# Autodesk Inventor assembly: DeviceForScheme
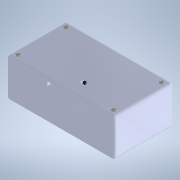
[picture p0: Inventor's stored thumbnail of the model, 180x180]
Saved by Autodesk Inventor 2022 (Build 260153000, 153)
## iProperties
Created: 2021-03-07
Part Number: DeviceForScheme
Description: STEP AP214
Document SubType Name: Assembly
Designer: user
Sending System: SolidWorks 2017
Preprocessor: SwSTEP 2.0
Title: Gainta G1098.STEP
Revision Number: ANY
## Documents named in this file (6)
- C:\Study\Diplom\case\DeviceForScheme.iam
- C:\Study\Diplom\case\Îñíîâàíèå.ipt
- C:\Study\Diplom\case\Êðûøêà.ipt
- C:\Study\Diplom\Altium\Diplom\Project Outputs for Diplom\InventorNew\PCBDiplomPCB.iam
- C:\Users\user\Documents\Inventor\Content Center Files\R2022\ru-RU\AS 1427(05)\AS 1427 - M2.5 x 16(5) II.ipt
- C:\Users\user\Documents\Inventor\Content Center Files\R2022\ru-RU\AS 1427(05)\AS 1427 - M3 x 5(5) II.ipt
## Components (11 placed, 5 different names)
1. Îñíîâàíèå_1 — Вставка:6
2. Êðûøêà_2 — Вставка:1, Вставка:4, Вставка:5, Вставка:6, Вставка:7, Вставка:8, Вставка:9, Вставка:10
3. PCBDiplomPCB:1 [sub-assembly] — Вставка:1, Вставка:2, Вставка:3
4. AS 1427 H - метрическая M2.5 x 16:1 — Вставка:8
5. AS 1427 H - метрическая M2.5 x 16:2 — Вставка:9
6. AS 1427 H - метрическая M2.5 x 16:3 — Вставка:7
7. AS 1427 H - метрическая M2.5 x 16:4 — Вставка:10
8. AS 1427 H - метрическая M3 x 5:1 — Вставка:3
9. AS 1427 H - метрическая M3 x 5:2 — Вставка:4
10. AS 1427 H - метрическая M3 x 5:3 — Вставка:5
11. AS 1427 H - метрическая M3 x 5:4 — Вставка:2
## Relationships (10: Insert 10)
- Вставка:1 [Insert]: Êðûøêà_2 ↔ PCBDiplomPCB:1
- Вставка:2 [Insert]: PCBDiplomPCB:1 ↔ AS 1427 H - метрическая M3 x 5:4
- Вставка:3 [Insert]: PCBDiplomPCB:1 ↔ AS 1427 H - метрическая M3 x 5:1
- Вставка:4 [Insert]: Êðûøêà_2 ↔ AS 1427 H - метрическая M3 x 5:2
- Вставка:5 [Insert]: Êðûøêà_2 ↔ AS 1427 H - метрическая M3 x 5:3
- Вставка:6 [Insert]: Îñíîâàíèå_1 ↔ Êðûøêà_2
- Вставка:7 [Insert]: Êðûøêà_2 ↔ AS 1427 H - метрическая M2.5 x 16:3
- Вставка:8 [Insert]: Êðûøêà_2 ↔ AS 1427 H - метрическая M2.5 x 16:1
- Вставка:9 [Insert]: Êðûøêà_2 ↔ AS 1427 H - метрическая M2.5 x 16:2
- Вставка:10 [Insert]: Êðûøêà_2 ↔ AS 1427 H - метрическая M2.5 x 16:4
